# Autodesk Inventor assembly: Extension Shelf Assembly
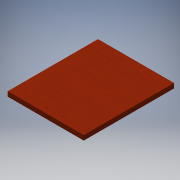
[picture p0: Inventor's stored thumbnail of the model, 180x180]
Saved by Autodesk Inventor 2016 (Build 200138000, 138)
## iProperties
Created: 2017-11-11
Part Number: Extension Shelf Assembly
Document SubType Name: Assembly
Designer: mathaetaes
Author: mathaetaes
## Documents named in this file (3)
- E:\Projects\3D Printer\printer projects\My Designs\Bar Cabinet\Extension Shelf Assembly.iam
- E:\Projects\3D Printer\printer projects\My Designs\Bar Cabinet\Extension Shelves.ipt
- E:\Projects\3D Printer\printer projects\My Designs\Bar Cabinet\hinge left.ipt
## Components (3 placed, 2 different names)
1. Extension Shelves:1 — Mate:1, Mate:2, Mate:3, Mate:4, Mate:5, Mate:6
2. hinge left:1 — Mate:1, Mate:5, Mate:6
3. hinge left:2 — Mate:2, Mate:3, Mate:4
## Relationships (6: Mate 6)
- Mate:1: Extension Shelves:1 ↔ hinge left:1
- Mate:2: Extension Shelves:1 ↔ hinge left:2
- Mate:3: Extension Shelves:1 ↔ hinge left:2
- Mate:4: Extension Shelves:1 ↔ hinge left:2
- Mate:5: Extension Shelves:1 ↔ hinge left:1
- Mate:6: Extension Shelves:1 ↔ hinge left:1
